# Autodesk Inventor assembly: Montagem Módulo Central
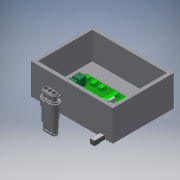
[picture p0: Inventor's stored thumbnail of the model, 180x180]
Saved by Autodesk Inventor 2019 (Build 230136000, 136)
## iProperties
Created: 2021-04-15
Part Number: Montagem Módulo Central
Document SubType Name: Assembly
Designer: luiza
Author: luiza
## Documents named in this file (6)
- G:\Meu Drive\Projetos\Projeto 2020 2021\Eletrônica 2020-2021\Projeção mecânica\Caixas\Módulo Central\Montagem Módulo Central.iam
- G:\Meu Drive\Projetos\Projeto 2020 2021\Eletrônica 2020-2021\Projeção elétrica\Placas\Placa Principal\[Cad] Placa Principal.ipt
- G:\Meu Drive\Projetos\Projeto 2020 2021\Eletrônica 2020-2021\Projeção mecânica\Caixas\Módulo Central\Base Modulo Central.ipt
- G:\Meu Drive\Projetos\Projeto 2020 2021\Eletrônica 2020-2021\Projeção mecânica\Caixas\Módulo Central\Dependencias\ublox NEO-6M.ipt
- G:\Meu Drive\Projetos\Projeto 2020 2021\Eletrônica 2020-2021\Projeção mecânica\Caixas\Módulo Central\Dependencias\ublox NEO-6M\Antenna.ipt
- G:\Meu Drive\Projetos\Projeto 2020 2021\Eletrônica 2020-2021\Projeção mecânica\Caixas\Módulo Central\AMP 3 position.ipt
## Components (5 placed, 5 different names)
1. [Cad] Placa Principal:1 — Mate:1, Mate:2, Mate:3
2. Antenna:1
3. ublox NEO-6M:1
4. Base Modulo Central:1
5. AMP 3 position:1
## Relationships (3: Mate 3)
- Mate:1 (-43.815 mm): [Cad] Placa Principal:1
- Mate:2 (-27.305 mm): [Cad] Placa Principal:1
- Mate:3: [Cad] Placa Principal:1
